# Autodesk Inventor assembly: gripper_testing
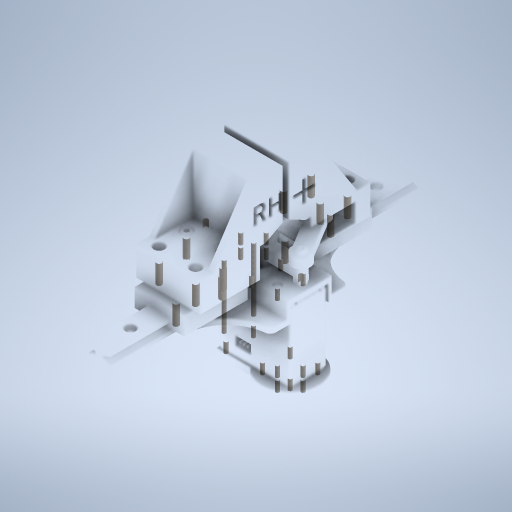
[picture p0: Inventor's stored thumbnail of the model, 512x512]
Saved by Autodesk Inventor 2024.2 (Build 282272000, 272)
## iProperties
Created: 2023-10-13
Part Number: gripper_testing
Document SubType Name: Assembly
Designer: 박동준
Author: 박동준
## Documents named in this file (20)
- C:\Users\chanh\내 드라이브\로봇\Humanoid\Roboin Humanoid Project\Inventor\rh_plus_7_axis_robot_arm_hardware\Assembly\3_Gripper.iam
- C:\Users\chanh\내 드라이브\로봇\Humanoid\Roboin Humanoid Project\Inventor\rh_plus_7_axis_robot_arm_hardware\Part\Frame\gripper\gripper.ipt
- C:\Users\chanh\내 드라이브\로봇\Humanoid\Roboin Humanoid Project\Inventor\rh_plus_7_axis_robot_arm_hardware\Part\Frame\gripper\gripper_base_frame.ipt
- C:\Users\chanh\내 드라이브\로봇\Humanoid\Roboin Humanoid Project\Inventor\rh_plus_7_axis_robot_arm_hardware\Part\Frame\axis_7_top_frame.ipt
- C:\Users\chanh\내 드라이브\로봇\Humanoid\Roboin Humanoid Project\Inventor\rh_plus_7_axis_robot_arm_hardware\Part\Frame\gripper\gripper_hand_connector.ipt
- C:\Users\chanh\내 드라이브\로봇\Humanoid\Roboin Humanoid Project\Inventor\rh_plus_7_axis_robot_arm_hardware\Part\Other Parts\lm_guide_cart.ipt
- C:\Users\chanh\내 드라이브\로봇\Humanoid\Roboin Humanoid Project\Inventor\rh_plus_7_axis_robot_arm_hardware\Part\Other Parts\lm_guide_rail.ipt
- C:\Users\chanh\내 드라이브\로봇\Humanoid\Roboin Humanoid Project\Inventor\rh_plus_7_axis_robot_arm_hardware\Part\HTD-45H, Horn\Horn\Top Horn.ipt
- C:\Users\chanh\내 드라이브\로봇\Humanoid\Roboin Humanoid Project\Inventor\rh_plus_7_axis_robot_arm_hardware\Part\Bolt, Bearing, Nut, Washer\M3x8.ipt
- C:\Users\chanh\내 드라이브\로봇\Humanoid\Roboin Humanoid Project\Inventor\rh_plus_7_axis_robot_arm_hardware\Part\Frame\axis_7_bottom_frame.ipt
- C:\Users\chanh\내 드라이브\로봇\Humanoid\Roboin Humanoid Project\Inventor\rh_plus_7_axis_robot_arm_hardware\Part\Bolt, Bearing, Nut, Washer\2030 Teflon Sheet.ipt
- C:\Users\chanh\내 드라이브\로봇\Humanoid\Roboin Humanoid Project\Inventor\rh_plus_7_axis_robot_arm_hardware\Part\Bolt, Bearing, Nut, Washer\M2x6 Round Bolt.ipt
- C:\Users\chanh\내 드라이브\로봇\Humanoid\Roboin Humanoid Project\Inventor\rh_plus_7_axis_robot_arm_hardware\Part\Bolt, Bearing, Nut, Washer\M3x10.ipt
- C:\Users\chanh\내 드라이브\로봇\Humanoid\Roboin Humanoid Project\Inventor\rh_plus_7_axis_robot_arm_hardware\Part\Bolt, Bearing, Nut, Washer\M3 Nylon Nut.ipt
- C:\Users\chanh\내 드라이브\로봇\Humanoid\Roboin Humanoid Project\Inventor\rh_plus_7_axis_robot_arm_hardware\Part\Bolt, Bearing, Nut, Washer\M3x16 Round Bolt.ipt
- C:\Users\chanh\내 드라이브\로봇\Humanoid\Roboin Humanoid Project\Inventor\rh_plus_7_axis_robot_arm_hardware\Part\Bolt, Bearing, Nut, Washer\M2x6 Bolt.ipt
- C:\Users\chanh\내 드라이브\로봇\Humanoid\Roboin Humanoid Project\Inventor\rh_plus_7_axis_robot_arm_hardware\Part\HTD-45H, Horn\Horn\M3x6.ipt
- C:\Users\chanh\내 드라이브\로봇\Humanoid\Roboin Humanoid Project\Inventor\rh_plus_7_axis_robot_arm_hardware\Part\Bolt, Bearing, Nut, Washer\M2x35 Round Bolt.ipt
- C:\Users\chanh\내 드라이브\로봇\Humanoid\Roboin Humanoid Project\Inventor\rh_plus_7_axis_robot_arm_hardware\Part\HTD-45H, Horn\HTD-45H\HTD-45H.ipt
- C:\Users\chanh\내 드라이브\로봇\Humanoid\Roboin Humanoid Project\Inventor\rh_plus_7_axis_robot_arm_hardware\Part\HTD-45H, Horn\HTD-45H\M2x32.ipt
## Components (55 placed, 19 different names)
1. M3x16 Round Bolt:1 — Rigid:56
2. M3x16 Round Bolt:2 — Rigid:57
3. M2x6 Bolt:1 — Rigid:36
4. M2x6 Bolt:2 — Rigid:37
5. M2x6 Bolt:3 — Rigid:38
6. M2x6 Bolt:4 — Rigid:39
7. M2x6 Round Bolt:1 — Rigid:2
8. M2x6 Round Bolt:2 — Rigid:4
9. M2x6 Round Bolt:3 — Rigid:6
10. M2x6 Round Bolt:4 — Rigid:11
11. M2x6 Round Bolt:5 — Rigid:3
12. M2x6 Round Bolt:6 — Rigid:7
13. M2x6 Round Bolt:7 — Rigid:8
14. M2x6 Round Bolt:8 — Rigid:5
15. M2x6 Round Bolt:9 — Rigid:10
16. M2x6 Round Bolt:10 — Rigid:9
17. M2x6 Round Bolt:11 — Rigid:54
18. M2x6 Round Bolt:12 — Rigid:52
19. M2x6 Round Bolt:13 — Rigid:53
20. M2x6 Round Bolt:14 — Rigid:55
21. M2x35 Round Bolt:2 — Rigid:50
22. M2x35 Round Bolt:4 — Rigid:51
23. M3x6:1 — Rigid:65
24. M3x8:1 — Rigid:59
25. M3x8:2 — Rigid:60
26. M3x8:3 — Rigid:62
27. M3x8:4 — Rigid:61
28. M3x8:5 — Mate:65, Mate:66
29. M3x8:6 — Mate:61, Mate:62
30. M3x8:7 — Mate:63, Mate:64
31. M3x8:8 — Mate:87, Mate:90, Mate:92
32. M3x8:9 — Mate:89, Mate:94, Mate:98
33. M3x8:10 — Mate:86, Mate:91, Mate:93
34. M3x10:1 — Rigid:22, Mate:102
35. M3x10:2 — Mate:88, Mate:95, Mate:101
36. M3 Nylon Nut:5 — Rigid:58
37. M3 Nylon Nut:6 — Rigid:63
38. M3 Nylon Nut:1 — Rigid:44
39. M3 Nylon Nut:4 — Rigid:45
40. gripper_base_frame:2 — Mate:81, Mate:82, Rigid:36, Rigid:37, Rigid:38, Rigid:39, Rigid:58, Rigid:63, Rigid:64
41. 2030 Teflon Sheet:1 — Rigid:12
42. axis_7_top_frame:1 — Mate:12, Mate:13, Mate:14, Mate:15, Mate:16, Mate:17, Rigid:48, Rigid:50, Rigid:51, Rigid:52, Rigid:53, Rigid:54, Rigid:55
43. axis_7_bottom_frame:1 — Rigid:2, Rigid:3, Rigid:4, Rigid:5, Rigid:6, Rigid:7, Rigid:8, Rigid:9, Rigid:10, Rigid:11, Rigid:12, Rigid:49
44. M2x32:1 — Rigid:47
45. M2x32:2 — Rigid:46
46. HTD-45H:1 — Rigid:46, Rigid:47, Rigid:48, Mate:103, Flush:1, Flush:2, Rigid:49, Rotational:1
47. Top Horn:1 — Rigid:64, Rigid:65, Rotational:1
48. gripper:1 — Angle:4, Mate:44, Mate:50, Mate:61, Mate:62, Mate:63, Mate:64, Mate:65, Mate:66, Rigid:22
49. gripper:2 — Angle:5, Mate:90, Mate:91, Mate:92, Mate:93, Mate:94, Mate:95, Mate:96, Mate:98
50. gripper_hand_connector:1 — Mate:81, Mate:101, Rigid:44, Rigid:56
51. gripper_hand_connector:2 — Mate:82, Mate:102, Rigid:45, Rigid:57
52. lm_guide_cart:1 — Mate:18, Angle:2, Mate:19, Mate:86, Mate:87, Mate:88, Mate:89, Angle:5, Mate:96
53. lm_guide_cart:2 — Mate:20, Angle:3, Mate:21, Angle:4, Mate:44, Mate:50
54. lm_guide_rail:1 — Mate:12, Mate:13, Mate:14, Mate:18, Angle:2, Mate:19, Rigid:59, Rigid:60
55. lm_guide_rail:2 — Mate:15, Mate:16, Mate:17, Mate:20, Angle:3, Mate:21, Rigid:61, Rigid:62
## Relationships (80: WeldJoint 38, Mate 35, Angle 4, Flush 2, RevoluteJoint 1)
- Rotational:1 [RevoluteJoint]: HTD-45H:1 ↔ Top Horn:1
- Mate:12: axis_7_top_frame:1 ↔ lm_guide_rail:1
- Mate:13: axis_7_top_frame:1 ↔ lm_guide_rail:1
- Mate:14: axis_7_top_frame:1 ↔ lm_guide_rail:1
- Mate:15: axis_7_top_frame:1 ↔ lm_guide_rail:2
- Mate:16: axis_7_top_frame:1 ↔ lm_guide_rail:2
- Mate:17: axis_7_top_frame:1 ↔ lm_guide_rail:2
- Mate:18: lm_guide_cart:1 ↔ lm_guide_rail:1
- Angle:2 (0 deg): lm_guide_cart:1 ↔ lm_guide_rail:1
- Mate:19: lm_guide_cart:1 ↔ lm_guide_rail:1
- Mate:20: lm_guide_cart:2 ↔ lm_guide_rail:2
- Angle:3 (0 deg): lm_guide_cart:2 ↔ lm_guide_rail:2
- Mate:21: lm_guide_cart:2 ↔ lm_guide_rail:2
- Angle:4 (0 deg): gripper:1 ↔ lm_guide_cart:2
- Rigid:59 [WeldJoint]: M3x8:1 ↔ lm_guide_rail:1
- Rigid:60 [WeldJoint]: M3x8:2 ↔ lm_guide_rail:1
- Rigid:61 [WeldJoint]: M3x8:4 ↔ lm_guide_rail:2
- Mate:44: gripper:1 ↔ lm_guide_cart:2
- Rigid:62 [WeldJoint]: M3x8:3 ↔ lm_guide_rail:2
- Rigid:2 [WeldJoint]: M2x6 Round Bolt:1 ↔ axis_7_bottom_frame:1
- Rigid:3 [WeldJoint]: M2x6 Round Bolt:5 ↔ axis_7_bottom_frame:1
- Rigid:4 [WeldJoint]: M2x6 Round Bolt:2 ↔ axis_7_bottom_frame:1
- Rigid:5 [WeldJoint]: M2x6 Round Bolt:8 ↔ axis_7_bottom_frame:1
- Rigid:6 [WeldJoint]: M2x6 Round Bolt:3 ↔ axis_7_bottom_frame:1
- Rigid:7 [WeldJoint]: M2x6 Round Bolt:6 ↔ axis_7_bottom_frame:1
- Rigid:8 [WeldJoint]: M2x6 Round Bolt:7 ↔ axis_7_bottom_frame:1
- Rigid:9 [WeldJoint]: M2x6 Round Bolt:10 ↔ axis_7_bottom_frame:1
- Rigid:10 [WeldJoint]: M2x6 Round Bolt:9 ↔ axis_7_bottom_frame:1
- Rigid:11 [WeldJoint]: M2x6 Round Bolt:4 ↔ axis_7_bottom_frame:1
- Rigid:12 [WeldJoint]: 2030 Teflon Sheet:1 ↔ axis_7_bottom_frame:1
- Mate:50: gripper:1 ↔ lm_guide_cart:2
- Mate:61: M3x8:6 ↔ gripper:1
- Mate:62: M3x8:6 ↔ gripper:1
- Mate:63: M3x8:7 ↔ gripper:1
- Mate:64: M3x8:7 ↔ gripper:1
- Mate:65: M3x8:5 ↔ gripper:1
- Mate:66: M3x8:5 ↔ gripper:1
- Mate:81: gripper_base_frame:2 ↔ gripper_hand_connector:1
- Mate:82: gripper_base_frame:2 ↔ gripper_hand_connector:2
- Rigid:22 [WeldJoint]: M3x10:1 ↔ gripper:1
- Mate:86: M3x8:10 ↔ lm_guide_cart:1
- Mate:87: M3x8:8 ↔ lm_guide_cart:1
- Mate:88: M3x10:2 ↔ lm_guide_cart:1
- Mate:89: M3x8:9 ↔ lm_guide_cart:1
- Angle:5 (0 deg): gripper:2 ↔ lm_guide_cart:1
- Mate:90: M3x8:8 ↔ gripper:2
- Mate:91: M3x8:10 ↔ gripper:2
- Mate:92: M3x8:8 ↔ gripper:2
- Mate:93: M3x8:10 ↔ gripper:2
- Mate:94: M3x8:9 ↔ gripper:2
- Mate:95: M3x10:2 ↔ gripper:2
- Mate:96: gripper:2 ↔ lm_guide_cart:1
- Mate:98: M3x8:9 ↔ gripper:2
- Rigid:36 [WeldJoint]: M2x6 Bolt:1 ↔ gripper_base_frame:2
- Rigid:37 [WeldJoint]: M2x6 Bolt:2 ↔ gripper_base_frame:2
- Rigid:38 [WeldJoint]: M2x6 Bolt:3 ↔ gripper_base_frame:2
- Rigid:39 [WeldJoint]: M2x6 Bolt:4 ↔ gripper_base_frame:2
- Mate:101: M3x10:2 ↔ gripper_hand_connector:1
- Mate:102: M3x10:1 ↔ gripper_hand_connector:2
- Rigid:44 [WeldJoint]: M3 Nylon Nut:1 ↔ gripper_hand_connector:1
- Rigid:45 [WeldJoint]: M3 Nylon Nut:4 ↔ gripper_hand_connector:2
- Rigid:46 [WeldJoint]: M2x32:2 ↔ HTD-45H:1
- Rigid:47 [WeldJoint]: M2x32:1 ↔ HTD-45H:1
- Rigid:48 [WeldJoint]: axis_7_top_frame:1 ↔ HTD-45H:1
- Mate:103: HTD-45H:1
- Flush:1: HTD-45H:1
- Flush:2: HTD-45H:1
- Rigid:49 [WeldJoint]: axis_7_bottom_frame:1 ↔ HTD-45H:1
- Rigid:50 [WeldJoint]: M2x35 Round Bolt:2 ↔ axis_7_top_frame:1
- Rigid:51 [WeldJoint]: M2x35 Round Bolt:4 ↔ axis_7_top_frame:1
- Rigid:52 [WeldJoint]: M2x6 Round Bolt:12 ↔ axis_7_top_frame:1
- Rigid:53 [WeldJoint]: M2x6 Round Bolt:13 ↔ axis_7_top_frame:1
- Rigid:54 [WeldJoint]: M2x6 Round Bolt:11 ↔ axis_7_top_frame:1
- Rigid:55 [WeldJoint]: M2x6 Round Bolt:14 ↔ axis_7_top_frame:1
- Rigid:56 [WeldJoint]: M3x16 Round Bolt:1 ↔ gripper_hand_connector:1
- Rigid:57 [WeldJoint]: M3x16 Round Bolt:2 ↔ gripper_hand_connector:2
- Rigid:58 [WeldJoint]: M3 Nylon Nut:5 ↔ gripper_base_frame:2
- Rigid:63 [WeldJoint]: M3 Nylon Nut:6 ↔ gripper_base_frame:2
- Rigid:64 [WeldJoint]: gripper_base_frame:2 ↔ Top Horn:1
- Rigid:65 [WeldJoint]: M3x6:1 ↔ Top Horn:1
